# Autodesk Inventor assembly: robot
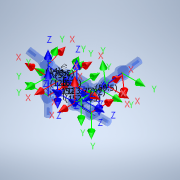
[picture p0: Inventor's stored thumbnail of the model, 180x180]
Saved by Autodesk Inventor 2020.2 (Build 242310000, 310)
## iProperties
Created: 2021-01-29
Part Number: robot
Document SubType Name: Assembly
Designer: DELL
Author: DELL
## Documents named in this file (7)
- D:\repo\experimental_flexipod\mesh\v7.0\robot.iam
- D:\repo\experimental_flexipod\mesh\v7.0\body.ipt
- D:\repo\experimental_flexipod\mesh\v7.0\hip.ipt
- D:\repo\experimental_flexipod\mesh\v7.0\thigh.ipt
- D:\repo\experimental_flexipod\mesh\v7.0\hip_back.ipt
- D:\repo\experimental_flexipod\mesh\v7.0\hip_back_mirror.ipt
- D:\repo\experimental_flexipod\mesh\v7.0\shank_2.ipt
## Components (13 placed, 6 different names)
1. body:1 — Flush:1, Flush:2, Flush:3, Mate:1, Mate:2, Mate:3, Mate:4, Mate:21, Mate:22, Mate:25, Mate:26, Angle:1, Angle:2, Angle:3, Angle:4, Angle:5, Angle:6, Angle:7, Angle:8
2. hip:1 — Mate:3, Mate:4, Mate:10, Mate:14, Angle:5
3. hip:2 — Mate:1, Mate:2, Mate:9, Flush:4, Angle:7
4. thigh:1 — Mate:9, Flush:4, Angle:8, Mate:30
5. thigh:2 — Mate:10, Mate:14, Mate:17, Angle:6
6. thigh:3 — Mate:16, Mate:24, Angle:2, Mate:29
7. thigh:4 — Mate:18, Mate:28, Angle:4, Flush:8
8. shank_2:1 — Mate:16
9. shank_2:2 — Mate:30
10. shank_2:3 — Mate:17
11. shank_2:4 — Mate:18
12. hip_back_mirror:1 — Mate:25, Mate:26, Mate:28, Angle:3, Flush:8
13. hip_back:1 — Mate:21, Mate:22, Mate:24, Angle:1, Mate:29
## Relationships (39: Mate 20, Angle 12, Flush 7)
- Flush:1: body:1
- Flush:2: body:1
- Flush:3: body:1
- Mate:1: body:1 ↔ hip:2
- Mate:2: body:1 ↔ hip:2
- Mate:3: body:1 ↔ hip:1
- Mate:4: body:1 ↔ hip:1
- Mate:9: hip:2 ↔ thigh:1
- Mate:10: hip:1 ↔ thigh:2
- Flush:4: hip:2 ↔ thigh:1
- Mate:14: hip:1 ↔ thigh:2
- Mate:16: thigh:3 ↔ shank_2:1
- Mate:17: thigh:2 ↔ shank_2:3
- Mate:18: thigh:4 ↔ shank_2:4
- [Mate]: thigh:4 ↔ shank_2:4
- [Flush]: thigh:3 ↔ shank_2:1
- [Flush]: thigh:2 ↔ shank_2:3
- [Mate]: thigh:1 ↔ shank_2:2
- Mate:21: body:1 ↔ hip_back:1
- Mate:22: body:1 ↔ hip_back:1
- Mate:24: thigh:3 ↔ hip_back:1
- Mate:25: body:1 ↔ hip_back_mirror:1
- Mate:26: body:1 ↔ hip_back_mirror:1
- Mate:28: thigh:4 ↔ hip_back_mirror:1
- Angle:1 (0 deg): body:1 ↔ hip_back:1
- Angle:2 (0 deg): body:1 ↔ thigh:3
- Angle:3 (0 deg): body:1 ↔ hip_back_mirror:1
- Angle:4 (0 deg): body:1 ↔ thigh:4
- Angle:5 (90 deg): body:1 ↔ hip:1
- Angle:6 (0 deg): body:1 ↔ thigh:2
- Angle:7 (0 deg): body:1 ↔ hip:2
- Angle:8 (0 deg): body:1 ↔ thigh:1
- [Angle] (0 deg): thigh:1 ↔ shank_2:2
- [Angle] (180 deg): thigh:2 ↔ shank_2:3
- [Angle] (0 deg): thigh:4 ↔ shank_2:4
- [Angle] (180 deg): thigh:3 ↔ shank_2:1
- Mate:29: thigh:3 ↔ hip_back:1
- Flush:8: thigh:4 ↔ hip_back_mirror:1
- Mate:30: thigh:1 ↔ shank_2:2
